# Autodesk Inventor assembly: Y_rail_Assembly_Rev3
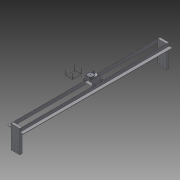
[picture p0: Inventor's stored thumbnail of the model, 180x180]
Saved by Autodesk Inventor 2015 (Build 190159000, 159)
## iProperties
Created: 2017-01-11
Part Number: Y_rail_Assembly_Rev3
Document SubType Name: Assembly
Designer: Guy
Author: Guy
## Documents named in this file (11)
- C:\Users\Guy\Documents\Fourth Year\Capstone\git\Capstone-Project\doc\CAD\LowLevel_Rev3\Y_rail_Assembly_Rev3.iam
- C:\Users\Guy\Documents\Fourth Year\Capstone\git\Capstone-Project\doc\CAD\LowLevel_Rev3\Y_Rail-SquareBar-Rev3.ipt
- C:\Users\Guy\Documents\Fourth Year\Capstone\git\Capstone-Project\doc\CAD\LowLevel_Rev3\Arm-SquareBar-Rev3.ipt
- C:\Users\Guy\Documents\Fourth Year\Capstone\git\Capstone-Project\doc\CAD\LowLevel_Rev3\XY_Wheel-SquareBar-Rev3.ipt
- C:\Users\Guy\Documents\Fourth Year\Capstone\git\Capstone-Project\doc\CAD\LowLevel_Rev3\EE_Base-SquareBar-Rev3.ipt
- C:\Users\Guy\Documents\Fourth Year\Capstone\git\Capstone-Project\doc\CAD\LowLevel_Rev3\Y_rail_Assembly_Rev3\Design Accelerator\Spur Gears1.iam
- C:\Users\Guy\Documents\Fourth Year\Capstone\git\Capstone-Project\doc\CAD\LowLevel_Rev3\Stepper_Motor_Holder-SquareBar-Rev3.ipt
- C:\Users\Guy\Documents\Fourth Year\Capstone\git\Capstone-Project\doc\CAD\Stepper Motor\NEMA 17\M1173041- NEMA 17.ipt
- C:\Users\Guy\Documents\Fourth Year\Capstone\git\Capstone-Project\doc\CAD\Nuts and Bolts\3-16in_1 1-4in_Bolt.ipt
- C:\Users\Guy\Documents\Fourth Year\Capstone\git\Capstone-Project\doc\CAD\Nuts and Bolts\3-16in_7-16in_washer(num8).ipt
- C:\Users\Guy\Documents\Fourth Year\Capstone\git\Capstone-Project\doc\CAD\Nuts and Bolts\3-16in_1-16in_nut(num2).ipt
## Components (24 placed, 10 different names)
1. Y_Rail-SquareBar-Rev3:1 — Mate:2, Mate:5, Mate:6, Tangent:1, Tangent:2, Mate:39
2. Y_Rail-SquareBar-Rev3:2 — Mate:1, Mate:4, Mate:7, Mate:8, Tangent:3, Tangent:4, Mate:12
3. Arm-SquareBar-Rev3:1 — Mate:1, Mate:2, Mate:5, Flush:1, Mate:7
4. Arm-SquareBar-Rev3:2 — Mate:4, Mate:6, Flush:1, Mate:8
5. XY_Wheel-SquareBar-Rev3:1 — Tangent:1, Mate:9, Flush:2, Mate:39, Mate:45, Mate:51
6. XY_Wheel-SquareBar-Rev3:2 — Tangent:4, Mate:9, Flush:4, Mate:15
7. XY_Wheel-SquareBar-Rev3:3 — Tangent:3, Mate:10, Mate:12, Flush:4, Mate:14, Mate:54, Mate:64, Mate:65
8. XY_Wheel-SquareBar-Rev3:4 — Tangent:2, Mate:10, Flush:2, Mate:13
9. Spur Gears:1 [sub-assembly] — Mate:17, Mate:36, Flush:5
10. EE_Base-SquareBar-Rev3:1 — Mate:13, Mate:14, Mate:15, Mate:17, Mate:37, Mate:38, Mate:53, Mate:55, Mate:63, Mate:66, Mate:67, Mate:68, Mate:69
11. M1173041- NEMA 17:1 — Mate:36, Flush:5, Mate:69, Mate:70
12. 3-16in_1 1-4in_Bolt:1 — Mate:37, Mate:38, Mate:44, Mate:46, Mate:48, Mate:49, Mate:52
13. 3-16in_7-16in_washer(num8):3 — Mate:44, Mate:45, Mate:47
14. 3-16in_1-16in_nut(num2):1 — Mate:46, Mate:47
15. 3-16in_7-16in_washer(num8):4 — Mate:48, Mate:50, Mate:51
16. 3-16in_1-16in_nut(num2):2 — Mate:49, Mate:50
17. 3-16in_1-16in_nut(num2):3 — Mate:52, Mate:53
18. 3-16in_1 1-4in_Bolt:2 — Mate:54, Mate:55, Mate:56, Mate:57, Mate:58, Mate:59, Mate:60
19. 3-16in_1-16in_nut(num2):4 — Mate:56, Mate:61
20. 3-16in_1-16in_nut(num2):5 — Mate:58, Mate:63
21. 3-16in_1-16in_nut(num2):6 — Mate:59, Mate:62
22. 3-16in_7-16in_washer(num8):5 — Mate:57, Mate:62, Mate:64
23. 3-16in_7-16in_washer(num8):6 — Mate:60, Mate:61, Mate:65
24. Stepper_Motor_Holder-SquareBar-Rev3:1 — Mate:66, Mate:67, Mate:68, Mate:70
## Relationships (53: Mate 45, Flush 4, Tangent 4)
- Mate:1: Y_Rail-SquareBar-Rev3:2 ↔ Arm-SquareBar-Rev3:1
- Mate:2: Y_Rail-SquareBar-Rev3:1 ↔ Arm-SquareBar-Rev3:1
- Mate:4: Y_Rail-SquareBar-Rev3:2 ↔ Arm-SquareBar-Rev3:2
- Mate:5: Y_Rail-SquareBar-Rev3:1 ↔ Arm-SquareBar-Rev3:1
- Mate:6: Y_Rail-SquareBar-Rev3:1 ↔ Arm-SquareBar-Rev3:2
- Flush:1: Arm-SquareBar-Rev3:1 ↔ Arm-SquareBar-Rev3:2
- Mate:7: Y_Rail-SquareBar-Rev3:2 ↔ Arm-SquareBar-Rev3:1
- Mate:8: Y_Rail-SquareBar-Rev3:2 ↔ Arm-SquareBar-Rev3:2
- Tangent:1: Y_Rail-SquareBar-Rev3:1 ↔ XY_Wheel-SquareBar-Rev3:1
- Tangent:2: Y_Rail-SquareBar-Rev3:1 ↔ XY_Wheel-SquareBar-Rev3:4
- Tangent:3: Y_Rail-SquareBar-Rev3:2 ↔ XY_Wheel-SquareBar-Rev3:3
- Tangent:4: Y_Rail-SquareBar-Rev3:2 ↔ XY_Wheel-SquareBar-Rev3:2
- Mate:9: XY_Wheel-SquareBar-Rev3:1 ↔ XY_Wheel-SquareBar-Rev3:2
- Mate:10: XY_Wheel-SquareBar-Rev3:3 ↔ XY_Wheel-SquareBar-Rev3:4
- Flush:2: XY_Wheel-SquareBar-Rev3:1 ↔ XY_Wheel-SquareBar-Rev3:4
- Mate:12 (1.75 mm): Y_Rail-SquareBar-Rev3:2 ↔ XY_Wheel-SquareBar-Rev3:3
- Flush:4: XY_Wheel-SquareBar-Rev3:2 ↔ XY_Wheel-SquareBar-Rev3:3
- Mate:13: XY_Wheel-SquareBar-Rev3:4 ↔ EE_Base-SquareBar-Rev3:1
- Mate:14: XY_Wheel-SquareBar-Rev3:3 ↔ EE_Base-SquareBar-Rev3:1
- Mate:15: XY_Wheel-SquareBar-Rev3:2 ↔ EE_Base-SquareBar-Rev3:1
- Mate:17: Spur Gears:1 ↔ EE_Base-SquareBar-Rev3:1
- Mate:36: Spur Gears:1 ↔ M1173041- NEMA 17:1
- Flush:5 (-10 mm): Spur Gears:1 ↔ M1173041- NEMA 17:1
- Mate:37: EE_Base-SquareBar-Rev3:1 ↔ 3-16in_1 1-4in_Bolt:1
- Mate:38: EE_Base-SquareBar-Rev3:1 ↔ 3-16in_1 1-4in_Bolt:1
- Mate:39: Y_Rail-SquareBar-Rev3:1 ↔ XY_Wheel-SquareBar-Rev3:1
- Mate:44: 3-16in_1 1-4in_Bolt:1 ↔ 3-16in_7-16in_washer(num8):3
- Mate:45: XY_Wheel-SquareBar-Rev3:1 ↔ 3-16in_7-16in_washer(num8):3
- Mate:46: 3-16in_1 1-4in_Bolt:1 ↔ 3-16in_1-16in_nut(num2):1
- Mate:47: 3-16in_7-16in_washer(num8):3 ↔ 3-16in_1-16in_nut(num2):1
- Mate:48: 3-16in_1 1-4in_Bolt:1 ↔ 3-16in_7-16in_washer(num8):4
- Mate:49: 3-16in_1 1-4in_Bolt:1 ↔ 3-16in_1-16in_nut(num2):2
- Mate:50: 3-16in_7-16in_washer(num8):4 ↔ 3-16in_1-16in_nut(num2):2
- Mate:51: XY_Wheel-SquareBar-Rev3:1 ↔ 3-16in_7-16in_washer(num8):4
- Mate:52: 3-16in_1 1-4in_Bolt:1 ↔ 3-16in_1-16in_nut(num2):3
- Mate:53: EE_Base-SquareBar-Rev3:1 ↔ 3-16in_1-16in_nut(num2):3
- Mate:54: XY_Wheel-SquareBar-Rev3:3 ↔ 3-16in_1 1-4in_Bolt:2
- Mate:55: EE_Base-SquareBar-Rev3:1 ↔ 3-16in_1 1-4in_Bolt:2
- Mate:56: 3-16in_1 1-4in_Bolt:2 ↔ 3-16in_1-16in_nut(num2):4
- Mate:57: 3-16in_1 1-4in_Bolt:2 ↔ 3-16in_7-16in_washer(num8):5
- Mate:58: 3-16in_1 1-4in_Bolt:2 ↔ 3-16in_1-16in_nut(num2):5
- Mate:59: 3-16in_1 1-4in_Bolt:2 ↔ 3-16in_1-16in_nut(num2):6
- Mate:60: 3-16in_1 1-4in_Bolt:2 ↔ 3-16in_7-16in_washer(num8):6
- Mate:61: 3-16in_1-16in_nut(num2):4 ↔ 3-16in_7-16in_washer(num8):6
- Mate:62: 3-16in_1-16in_nut(num2):6 ↔ 3-16in_7-16in_washer(num8):5
- Mate:63: EE_Base-SquareBar-Rev3:1 ↔ 3-16in_1-16in_nut(num2):5
- Mate:64: XY_Wheel-SquareBar-Rev3:3 ↔ 3-16in_7-16in_washer(num8):5
- Mate:65: XY_Wheel-SquareBar-Rev3:3 ↔ 3-16in_7-16in_washer(num8):6
- Mate:66: EE_Base-SquareBar-Rev3:1 ↔ Stepper_Motor_Holder-SquareBar-Rev3:1
- Mate:67: EE_Base-SquareBar-Rev3:1 ↔ Stepper_Motor_Holder-SquareBar-Rev3:1
- Mate:68: EE_Base-SquareBar-Rev3:1 ↔ Stepper_Motor_Holder-SquareBar-Rev3:1
- Mate:69: EE_Base-SquareBar-Rev3:1 ↔ M1173041- NEMA 17:1
- Mate:70: M1173041- NEMA 17:1 ↔ Stepper_Motor_Holder-SquareBar-Rev3:1
